# Autodesk Inventor assembly: Right Bearing Flat NScrew Slotted Offset
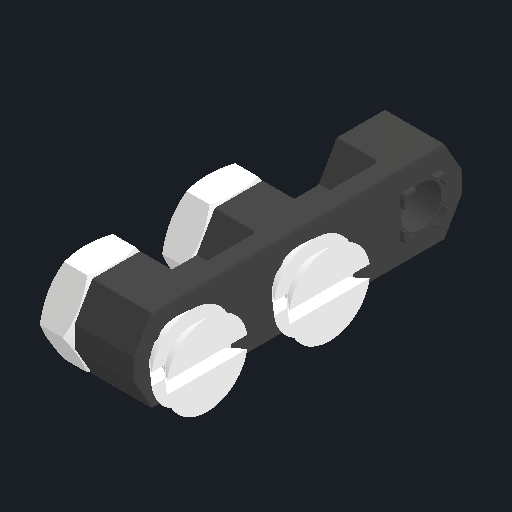
[picture p0: Inventor's stored thumbnail of the model, 512x512]
Saved by Autodesk Inventor 2025 (Build 290162000, 162)
## iProperties
Created: 2024-10-10
Part Number: Right Bearing Flat NScrew Slotted Offset
Document SubType Name: Assembly
Designer: Averey Ku
Author: Averey Ku
## Documents named in this file (5)
- D:\VEX\High Stakes\CAD\V2\Intake\Right Angle Structure\Right Bearing Flat NScrew Slotted Offset.iam
- D:\VEX\High Stakes\CAD\V2\Intake\Right Angle Structure\Right NScrew Slotted Threaded .500.ipt
- D:\VEX\High Stakes\CAD\V2\Intake\Right Angle Structure\Right Bearing Flat Low Profile.ipt
- D:\VEX\High Stakes\CAD\ROBOPROS-CAD-Inventor\Structure\Hardware\Nut Nylon\Nut Nylon - White.ipt
- D:\VEX\High Stakes\CAD\ROBOPROS-CAD-Inventor\Structure\Hardware\Nut Nylon.ipt
## Components (7 placed, 3 different names)
1. Right NScrew Slotted Threaded .500:1 — Insert:5, Insert:7
2. Right NScrew Slotted Threaded .500:2 — Insert:2, Insert:8
3. Right Bearing Flat Low Profile:1 — Insert:2, Insert:5, Insert:4, Insert:6
4. Nut Nylon - White:1 — Insert:4
5. Nut Nylon - White:2 — Insert:6
6. Right NScrew Slotted Threaded .500:3 — Insert:8
7. Right NScrew Slotted Threaded .500:4 — Insert:7
## Relationships (6: Insert 6)
- Insert:2 (-1.5875 mm): Right NScrew Slotted Threaded .500:2 ↔ Right Bearing Flat Low Profile:1
- Insert:5 (-1.5875 mm): Right NScrew Slotted Threaded .500:1 ↔ Right Bearing Flat Low Profile:1
- Insert:4 (1.27 mm): Right Bearing Flat Low Profile:1 ↔ Nut Nylon - White:1
- Insert:6 (1.27 mm): Right Bearing Flat Low Profile:1 ↔ Nut Nylon - White:2
- Insert:8 (-1.5875 mm): Right NScrew Slotted Threaded .500:2 ↔ Right NScrew Slotted Threaded .500:3
- Insert:7 (-1.5875 mm): Right NScrew Slotted Threaded .500:1 ↔ Right NScrew Slotted Threaded .500:4
